# Autodesk Inventor assembly: Main Assembly
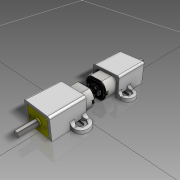
[picture p0: Inventor's stored thumbnail of the model, 180x180]
Saved by Autodesk Inventor 2013 SP2 (Build 170200200, 200)
## iProperties
Created: 2014-04-15
Part Number: Main Assembly
Document SubType Name: Assembly
Designer: Kevin
Author: Kevin
## Documents named in this file (3)
- C:\Users\Kevin\Dropbox\IEEEUCR-MM-2014\hardware\Reference_Mouse_v2\3D\Main Assembly.iam
- C:\Users\Kevin\Dropbox\IEEEUCR-MM-2014\hardware\Reference_Mouse_v2\3D\Pololu Micro Metal Gearmotor Bracket Extended.ipt
- C:\Users\Kevin\Dropbox\IEEEUCR-MM-2014\hardware\Reference_Mouse_v2\3D\Pololu Metal Gearmotor.ipt
## Components (4 placed, 2 different names)
1. Pololu Micro Metal Gearmotor Bracket Extended:1 — Mate:1, Mate:2, Flush:1, Mate:3, Flush:2, Flush:3
2. Pololu Metal Gearmotor:1 — Mate:1, Mate:2, Flush:1
3. Pololu Micro Metal Gearmotor Bracket Extended:2 — Mate:3, Flush:2, Flush:3, Mate:4, Flush:4, Mate:5
4. Pololu Metal Gearmotor:2 — Mate:4, Flush:4, Mate:5
## Relationships (9: Mate 5, Flush 4)
- Mate:1: Pololu Micro Metal Gearmotor Bracket Extended:1 ↔ Pololu Metal Gearmotor:1
- Mate:2: Pololu Micro Metal Gearmotor Bracket Extended:1 ↔ Pololu Metal Gearmotor:1
- Flush:1: Pololu Micro Metal Gearmotor Bracket Extended:1 ↔ Pololu Metal Gearmotor:1
- Mate:3 (19.05 mm): Pololu Micro Metal Gearmotor Bracket Extended:1 ↔ Pololu Micro Metal Gearmotor Bracket Extended:2
- Flush:2: Pololu Micro Metal Gearmotor Bracket Extended:1 ↔ Pololu Micro Metal Gearmotor Bracket Extended:2
- Flush:3: Pololu Micro Metal Gearmotor Bracket Extended:1 ↔ Pololu Micro Metal Gearmotor Bracket Extended:2
- Mate:4: Pololu Micro Metal Gearmotor Bracket Extended:2 ↔ Pololu Metal Gearmotor:2
- Flush:4: Pololu Micro Metal Gearmotor Bracket Extended:2 ↔ Pololu Metal Gearmotor:2
- Mate:5: Pololu Micro Metal Gearmotor Bracket Extended:2 ↔ Pololu Metal Gearmotor:2
